# Autodesk Inventor assembly: Motor
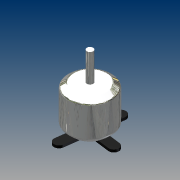
[picture p0: Inventor's stored thumbnail of the model, 180x180]
Saved by Autodesk Inventor 2013 (Build 170138000, 138)
## iProperties
Created: 2011-07-19
Part Number: Motor
Document SubType Name: Assembly
Designer: Nathan
Author: Nathan
## Documents named in this file (3)
- C:\Users\Nathan\Desktop\Dropbox\Quadcopter\Motor.iam
- C:\Users\Nathan\Desktop\Dropbox\Quadcopter\MotorTop.ipt
- C:\Users\Nathan\Desktop\Dropbox\Quadcopter\MotorBottom.ipt
## Components (2 placed, 2 different names)
1. MotorTop:1 — Mate:1, Mate:2
2. MotorBottom:1 — Mate:1, Mate:2
## Relationships (2: Mate 2)
- Mate:1: MotorTop:1 ↔ MotorBottom:1
- Mate:2: MotorTop:1 ↔ MotorBottom:1
